# Autodesk Inventor assembly: 组装
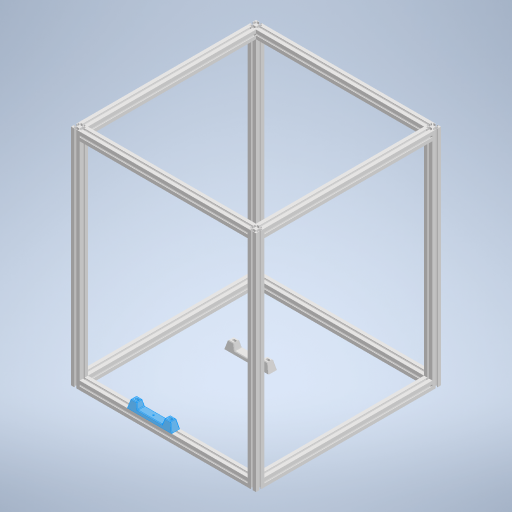
[picture p0: Inventor's stored thumbnail of the model, 512x512]
Saved by Autodesk Inventor 2023 (Build 270158000, 158)
## iProperties
Created: 2022-04-16
Part Number: 组装
Document SubType Name: Assembly
Designer: Zhong
Author: Zhong
## Documents named in this file (4)
- F:\成品\建模\3D打印机\3d打印机完整\组装.iam
- F:\成品\建模\3D打印机\3030型材\3030型材.ipt
- F:\成品\建模\3D打印机\3030型材\3030型材-600mm.ipt
- F:\成品\建模\3D打印机\Z光轴固定\Z光轴固定.ipt
## Components (14 placed, 3 different names)
1. Z光轴固定:1 — 配合:1, 配合:2
2. Z光轴固定:2
3. 3030型材:1 — 刚性:1, 刚性:3, 刚性:10, 刚性:11
4. 3030型材:2 — 刚性:2
5. 3030型材:3 — 刚性:6, 刚性:7, 刚性:8, 刚性:9
6. 3030型材:4 — 刚性:4, 刚性:5
7. 3030型材-600mm:1 — 刚性:3, 刚性:4
8. 3030型材-600mm:2 — 刚性:1, 刚性:2
9. 3030型材-600mm:3 — 刚性:7
10. 3030型材-600mm:4 — 刚性:5, 刚性:6
11. 3030型材-600mm:5 — 刚性:10
12. 3030型材-600mm:6 — 刚性:11
13. 3030型材-600mm:7 — 刚性:8, 配合:1, 配合:2
14. 3030型材-600mm:8 — 刚性:9
## Relationships (13: WeldJoint 11, Mate 2)
- 刚性:1 [WeldJoint]: 3030型材:1 ↔ 3030型材-600mm:2
- 刚性:2 [WeldJoint]: 3030型材:2 ↔ 3030型材-600mm:2
- 刚性:3 [WeldJoint]: 3030型材:1 ↔ 3030型材-600mm:1
- 刚性:4 [WeldJoint]: 3030型材:4 ↔ 3030型材-600mm:1
- 刚性:5 [WeldJoint]: 3030型材:4 ↔ 3030型材-600mm:4
- 刚性:6 [WeldJoint]: 3030型材:3 ↔ 3030型材-600mm:4
- 刚性:7 [WeldJoint]: 3030型材:3 ↔ 3030型材-600mm:3
- 刚性:8 [WeldJoint]: 3030型材:3 ↔ 3030型材-600mm:7
- 刚性:9 [WeldJoint]: 3030型材:3 ↔ 3030型材-600mm:8
- 刚性:10 [WeldJoint]: 3030型材:1 ↔ 3030型材-600mm:5
- 刚性:11 [WeldJoint]: 3030型材:1 ↔ 3030型材-600mm:6
- 配合:1 [Mate]: Z光轴固定:1 ↔ 3030型材-600mm:7
- 配合:2 [Mate] (-1 mm): Z光轴固定:1 ↔ 3030型材-600mm:7
